# Autodesk Inventor assembly: case
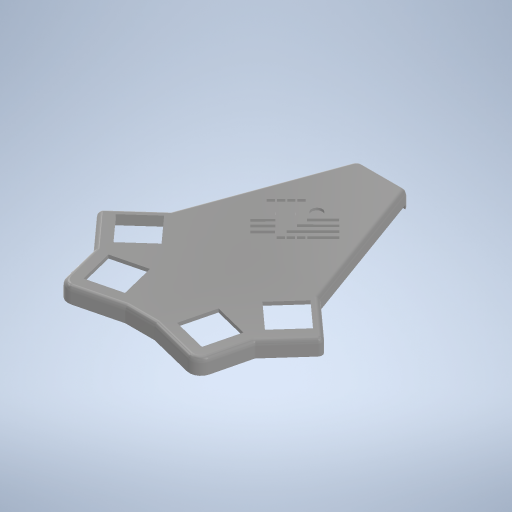
[picture p0: Inventor's stored thumbnail of the model, 512x512]
Saved by Autodesk Inventor 2024 (Build 280153000, 153)
## iProperties
Created: 2024-09-29
Part Number: case
Document SubType Name: Assembly
Designer: nikla
Author: nikla
## Documents named in this file (6)
- C:\Users\nikla\OneDrive\Keyboards\Blavinge\case\1-part\top.iam
- C:\Users\nikla\OneDrive\Keyboards\Blavinge\kicad\blavinge\blavinge.iam
- C:\Users\nikla\OneDrive\Keyboards\Blavinge\case\1-part\middle_top.ipt
- C:\Users\nikla\OneDrive\Keyboards\Blavinge\case\1-part\left_top.ipt
- C:\Users\nikla\OneDrive\Keyboards\Blavinge\case\1-part\left_top_MIR.ipt
- C:\Users\nikla\OneDrive\Keyboards\Blavinge\case\1-part\top.ipt
## Components (5 placed, 5 different names)
1. blavinge:1 [sub-assembly] — Fluchtend:1, Fluchtend:3, Fluchtend:4
2. middle_top:1 — Fluchtend:1, Fluchtend:5
3. left_top:1 — Fluchtend:3, Fluchtend:4
4. left_top_MIR:1
5. top:1 — Fluchtend:5
## Relationships (4: Flush 4)
- Fluchtend:1 [Flush]: blavinge:1 ↔ middle_top:1
- Fluchtend:3 [Flush]: blavinge:1 ↔ left_top:1
- Fluchtend:4 [Flush]: blavinge:1 ↔ left_top:1
- Fluchtend:5 [Flush]: middle_top:1 ↔ top:1
